# Autodesk Inventor assembly: Assemby 3
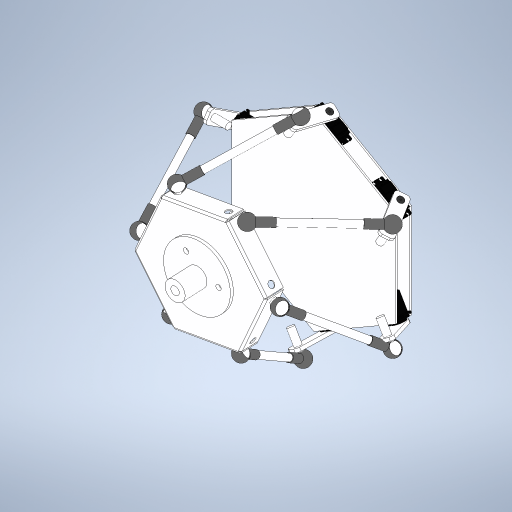
[picture p0: Inventor's stored thumbnail of the model, 512x512]
Saved by Autodesk Inventor 2023 (Build 270158000, 158)
## iProperties
Created: 2022-06-30
Part Number: Assemby 3
Document SubType Name: Assembly
Designer: earls
Mass: 2042.22 g
Surface Area: 5210.5 cm^2
Volume: 756.378 cm^3
Density: 2.7 g/cm^3
Author: earls
## Documents named in this file (12)
- C:\Users\earls\Documents\stewart-platform\CAD\Assemby 3.iam
- C:\Users\earls\Documents\stewart-platform\CAD\Stewart Assembly.iam
- C:\Users\earls\Documents\stewart-platform\CAD\Moving platform.ipt
- C:\Users\earls\Documents\stewart-platform\CAD\Spherical joint\Part2.ipt
- C:\Users\earls\Documents\stewart-platform\CAD\Spherical joint\Part1.ipt
- C:\Users\earls\Documents\stewart-platform\CAD\Rod qty-6.ipt
- C:\Users\earls\Documents\stewart-platform\CAD\Test flange.ipt
- C:\Users\earls\Documents\stewart-platform\CAD\Assemby 3\AIP\FEA\e0qqxsw9s.fins
- C:\Users\earls\Documents\stewart-platform\CAD\Assemby 3\AIP\FEA\e0qqxsw9s.fsat
- C:\Users\earls\Documents\stewart-platform\CAD\Assemby 3\AIP\FEA\e0qqxswao.ftes
- C:\Users\earls\Documents\stewart-platform\CAD\Assemby 3\AIP\FEA\e0qqxswao.fwiz
- C:\Users\earls\Documents\stewart-platform\CAD\Assemby 3\AIP\FEA\e0qqxswo0.fmsh
## Components (33 placed, 6 different names)
1. Stewart Assembly:1 [sub-assembly] — Insert:1, Insert:4, Insert:5, Insert:7, Insert:10, Insert:12
2. Moving platform:1 — Insert:2, Insert:3, Insert:6, Insert:8, Insert:9, Insert:11, Mate:25, Mate:26
3. Part2:1 — Insert:2, Ball:1
4. Part2:2 — Insert:1, Ball:2
5. Part1:1 — Ball:2, Mate:3, Mate:4
6. Part1:2 — Ball:1, Mate:5, Mate:6
7. Rod qty-6:1 — Mate:3, Mate:4, Mate:5, Mate:6
8. Rod qty-6:2 — Mate:7, Mate:8, Mate:9
9. Part1:3 — Ball:3, Mate:9
10. Part2:3 — Insert:3, Ball:3
11. Part2:4 — Insert:4, Ball:4
12. Part1:4 — Ball:4, Mate:7, Mate:8
13. Part1:5 — Ball:5, Mate:10, Mate:11
14. Part2:5 — Insert:5, Ball:5
15. Part1:6 — Ball:6, Mate:12, Mate:13
16. Part2:6 — Insert:6, Ball:6
17. Rod qty-6:3 — Mate:10, Mate:11, Mate:12, Mate:13
18. Part1:7 — Ball:8, Mate:16, Mate:24
19. Part2:7 — Insert:8, Ball:8
20. Part1:8 — Ball:7, Mate:14, Mate:15
21. Part2:8 — Insert:7, Ball:7
22. Rod qty-6:4 — Mate:14, Mate:15, Mate:16, Mate:24
23. Part1:9 — Ball:9, Mate:18, Mate:19
24. Part2:9 — Insert:9, Ball:9
25. Part1:10 — Ball:10, Mate:17, Mate:23
26. Part2:10 — Insert:10, Ball:10
27. Rod qty-6:5 — Mate:17, Mate:18, Mate:19, Mate:23
28. Part1:11 — Ball:11, Mate:21, Mate:22
29. Part2:11 — Insert:11, Ball:11
30. Part1:12 — Ball:12, Mate:20
31. Part2:12 — Insert:12, Ball:12
32. Rod qty-6:6 — Mate:20, Mate:21, Mate:22
33. Test flange:1 — Mate:25, Mate:26
## Relationships (48: Mate 24, Insert 12, BallJoint 12)
- Insert:1 (-3 mm): Stewart Assembly:1 ↔ Part2:2
- Insert:2 (-3 mm): Moving platform:1 ↔ Part2:1
- Ball:1: Part2:1 ↔ Part1:2
- Ball:2: Part2:2 ↔ Part1:1
- Mate:3: Part1:1 ↔ Rod qty-6:1
- Mate:4: Part1:1 ↔ Rod qty-6:1
- Mate:5: Part1:2 ↔ Rod qty-6:1
- Mate:6: Part1:2 ↔ Rod qty-6:1
- Insert:3 (-3 mm): Moving platform:1 ↔ Part2:3
- Ball:3: Part1:3 ↔ Part2:3
- Insert:4 (-3 mm): Stewart Assembly:1 ↔ Part2:4
- Ball:4: Part2:4 ↔ Part1:4
- Mate:7: Rod qty-6:2 ↔ Part1:4
- Mate:8: Rod qty-6:2 ↔ Part1:4
- Mate:9: Rod qty-6:2 ↔ Part1:3
- Insert:5 (-3 mm): Stewart Assembly:1 ↔ Part2:5
- Insert:6 (-3 mm): Moving platform:1 ↔ Part2:6
- Ball:5: Part1:5 ↔ Part2:5
- Ball:6: Part1:6 ↔ Part2:6
- Mate:10: Part1:5 ↔ Rod qty-6:3
- Mate:11: Part1:5 ↔ Rod qty-6:3
- Mate:12: Part1:6 ↔ Rod qty-6:3
- Mate:13: Part1:6 ↔ Rod qty-6:3
- Insert:7 (-3 mm): Stewart Assembly:1 ↔ Part2:8
- Insert:8 (-3 mm): Moving platform:1 ↔ Part2:7
- Ball:7: Part1:8 ↔ Part2:8
- Ball:8: Part1:7 ↔ Part2:7
- Mate:14: Part1:8 ↔ Rod qty-6:4
- Mate:15: Part1:8 ↔ Rod qty-6:4
- Mate:16: Part1:7 ↔ Rod qty-6:4
- Insert:9 (-3 mm): Moving platform:1 ↔ Part2:9
- Ball:9: Part1:9 ↔ Part2:9
- Insert:10 (-3 mm): Stewart Assembly:1 ↔ Part2:10
- Ball:10: Part1:10 ↔ Part2:10
- Mate:17: Part1:10 ↔ Rod qty-6:5
- Mate:18: Part1:9 ↔ Rod qty-6:5
- Mate:19: Part1:9 ↔ Rod qty-6:5
- Insert:11 (-3 mm): Moving platform:1 ↔ Part2:11
- Insert:12 (-3 mm): Stewart Assembly:1 ↔ Part2:12
- Ball:11: Part1:11 ↔ Part2:11
- Ball:12: Part1:12 ↔ Part2:12
- Mate:20: Part1:12 ↔ Rod qty-6:6
- Mate:21: Part1:11 ↔ Rod qty-6:6
- Mate:22: Part1:11 ↔ Rod qty-6:6
- Mate:23: Part1:10 ↔ Rod qty-6:5
- Mate:24: Part1:7 ↔ Rod qty-6:4
- Mate:25: Moving platform:1 ↔ Test flange:1
- Mate:26: Moving platform:1 ↔ Test flange:1
## Named parameters: sa_0 = 10000, sa_1 = 1962, sa_2 = 0, sa_3 = 0, sa_4 = 0, sa_5 = 0, sa_6 = 0, sa_7 = 0, sa_8 = 0, sa_9 = 0, sa_10 = 0, sa_11 = 0, sa_12 = 0, sa_13 = 0, sa_26 = 0, sa_27 = 0, sa_28 = 0, sa_29 = 0, sa_30 = 0, sa_31 = 0, sa_32 = 0, sa_33 = 0, sa_34 = 0, sa_35 = 0, sa_36 = 0, sa_37 = 0, sa_38 = 0, sa_39 = 0, sa_40 = 0, sa_41 = 0, sa_42 = 0, sa_43 = 0, sa_46 = 0, sa_47 = 0, sa_48 = 0, sa_49 = 0, sa_50 = 0, sa_51 = 0, sa_52 = 0, sa_53 = 0, sa_54 = 0, sa_55 = 0, sa_56 = 0, sa_57 = 0, sa_58 = 0, sa_59 = 0, sa_60 = 0, sa_61 = 0, sa_62 = 0, sa_63 = 0, sa_64 = 0, sa_65 = 0, sa_66 = 0, sa_67 = 0, sa_68 = 0, sa_69 = 0, sa_70 = 0, sa_71 = 0, sa_72 = 0, sa_73 = 0, sa_74 = 0, sa_75 = 0, sa_76 = 0, sa_77 = 0, sa_78 = 0, sa_79 = 0, sa_80 = 0, sa_81 = 0, sa_82 = 0, sa_83 = 0, sa_84 = 0, sa_85 = 0, sa_86 = 0, sa_87 = 0, sa_88 = 0, sa_89 = 0, sa_90 = 0, sa_91 = 0, sa_92 = 0, sa_93 = 0, sa_94 = 0, sa_95 = 0, sa_96 = 0, sa_97 = 0, sa_98 = 0, sa_99 = 0, sa_100 = 0, sa_101 = 0, sa_102 = 0, sa_103 = 0, sa_104 = 0, sa_105 = 0, sa_106 = 0, sa_107 = 0, sa_108 = 0, sa_109 = 0, sa_110 = 0, sa_111 = 0, sa_112 = 0, sa_113 = 0, sa_114 = 0, sa_115 = 0, sa_116 = 0, sa_117 = 0, sa_118 = 0, sa_119 = 0, sa_120 = 0, sa_121 = 0, sa_122 = 0, sa_123 = 0, sa_124 = 0, sa_125 = 0, sa_126 = 0, sa_127 = 0, sa_128 = 1962, sa_129 = 981, sa_130 = 196.2, sa_131 = 0, sa_132 = 0, sa_133 = 0, sa_134 = 0, sa_135 = 0, sa_136 = 0, sa_137 = 0, sa_138 = 0, sa_139 = 0, sa_140 = 0, sa_141 = 0, sa_142 = 0, sa_143 = 0, sa_144 = 0, sa_145 = 0, sa_146 = 0, sa_147 = 0, sa_148 = 0, sa_149 = 0, sa_150 = 0, sa_151 = 0, sa_152 = 0, sa_153 = 0, sa_154 = 0
note: some values were not read from the file. Shown as the stored number, unit unknown: "sa_0", "sa_1", "sa_2", "sa_3", "sa_4", "sa_5", "sa_6", "sa_7", "sa_8", "sa_9", "sa_10", "sa_11", "sa_12", "sa_13", "sa_26", "sa_27", "sa_28", "sa_29", "sa_30", "sa_31", "sa_32", "sa_33", "sa_34", "sa_35", "sa_36", "sa_37", "sa_38", "sa_39", "sa_40", "sa_41", "sa_42", "sa_43", "sa_46", "sa_47", "sa_48", "sa_49", "sa_50", "sa_51", "sa_52", "sa_53", "sa_54", "sa_55", "sa_56", "sa_57", "sa_58", "sa_59", "sa_60", "sa_61", "sa_62", "sa_63", "sa_64", "sa_65", "sa_66", "sa_67", "sa_68", "sa_69", "sa_70", "sa_71", "sa_72", "sa_73", "sa_74", "sa_75", "sa_76", "sa_77", "sa_78", "sa_79", "sa_80", "sa_81", "sa_82", "sa_83", "sa_84", "sa_85", "sa_86", "sa_87", "sa_88", "sa_89", "sa_90", "sa_91", "sa_92", "sa_93", "sa_94", "sa_95", "sa_96", "sa_97", "sa_98", "sa_99", "sa_100", "sa_101", "sa_102", "sa_103", "sa_104", "sa_105", "sa_106", "sa_107", "sa_108", "sa_109", "sa_110", "sa_111", "sa_112", "sa_113", "sa_114", "sa_115", "sa_116", "sa_117", "sa_118", "sa_119", "sa_120", "sa_121", "sa_122", "sa_123", "sa_124", "sa_125", "sa_126", "sa_127", "sa_128", "sa_129", "sa_130", "sa_131", "sa_132", "sa_133", "sa_134", "sa_135", "sa_136", "sa_137", "sa_138", "sa_139", "sa_140", "sa_141", "sa_142", "sa_143", "sa_144", "sa_145", "sa_146", "sa_147", "sa_148", "sa_149", "sa_150", "sa_151", "sa_152", "sa_153", "sa_154".
